# Autodesk Inventor assembly: smDriverStation-ver1-1111-2021
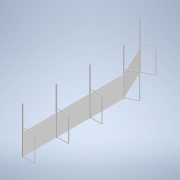
[picture p0: Inventor's stored thumbnail of the model, 180x180]
Saved by Autodesk Inventor 2021 (Build 250183000, 183)
## iProperties
Created: 2021-03-02
Part Number: smDriverStation-ver1-1111-2021
Document SubType Name: Assembly
Designer: CMurray
Author: CMurray
## Documents named in this file (3)
- F:\PHRC CADD 2021\2021 Game Design Challenge\Player Station\Assemblies\smDriverStation-ver1-1111-2021.iam
- F:\PHRC CADD 2021\2021 Game Design Challenge\Player Station\Parts\StationBase-ver2-1111-2021.ipt
- F:\PHRC CADD 2021\2021 Game Design Challenge\Player Station\Parts\StationDivider-ver1-1111-2021.iam
## Components (9 placed, 2 different names)
1. StationBase-ver2-1111-2021:2 — Mate:1, Flush:1, Flush:2, Mate:2, Flush:3, Flush:4, Flush:9, Flush:10
2. StationDivider-ver1-1111-2021:3 [sub-assembly] — Mate:1, Flush:1, Flush:2
3. StationDivider-ver1-1111-2021:4 [sub-assembly] — Mate:2, Flush:3, Flush:4, Mate:5
4. StationBase-ver2-1111-2021:3 — Flush:9, Flush:10, Mate:5, Flush:11, Flush:12
5. StationDivider-ver1-1111-2021:6 [sub-assembly] — Mate:6
6. StationBase-ver2-1111-2021:4 — Flush:11, Flush:12, Mate:6, Mate:7, Flush:13, Angle:1, Flush:14
7. StationDivider-ver1-1111-2021:7 [sub-assembly] — Mate:7, Flush:13, Mate:8, Angle:2
8. StationBase-ver2-1111-2021:5 — Mate:8, Angle:1, Flush:14, Mate:9, Flush:15, Flush:16
9. StationDivider-ver1-1111-2021:8 [sub-assembly] — Mate:9, Flush:15, Flush:16, Angle:2
## Relationships (24: Flush 14, Mate 8, Angle 2)
- Mate:1: StationBase-ver2-1111-2021:2 ↔ StationDivider-ver1-1111-2021:3
- Flush:1: StationBase-ver2-1111-2021:2 ↔ StationDivider-ver1-1111-2021:3
- Flush:2: StationBase-ver2-1111-2021:2 ↔ StationDivider-ver1-1111-2021:3
- Mate:2: StationBase-ver2-1111-2021:2 ↔ StationDivider-ver1-1111-2021:4
- Flush:3: StationBase-ver2-1111-2021:2 ↔ StationDivider-ver1-1111-2021:4
- Flush:4: StationBase-ver2-1111-2021:2 ↔ StationDivider-ver1-1111-2021:4
- [Mate]: StationBase-ver2-1111-2021:3 ↔ StationDivider-ver1-1111-2021:6
- [Flush]: StationBase-ver2-1111-2021:3 ↔ StationDivider-ver1-1111-2021:6
- [Flush]: StationBase-ver2-1111-2021:3 ↔ StationDivider-ver1-1111-2021:6
- Flush:9: StationBase-ver2-1111-2021:2 ↔ StationBase-ver2-1111-2021:3
- Flush:10: StationBase-ver2-1111-2021:2 ↔ StationBase-ver2-1111-2021:3
- Mate:5: StationDivider-ver1-1111-2021:4 ↔ StationBase-ver2-1111-2021:3
- Flush:11: StationBase-ver2-1111-2021:3 ↔ StationBase-ver2-1111-2021:4
- Flush:12: StationBase-ver2-1111-2021:3 ↔ StationBase-ver2-1111-2021:4
- Mate:6: StationDivider-ver1-1111-2021:6 ↔ StationBase-ver2-1111-2021:4
- Mate:7: StationBase-ver2-1111-2021:4 ↔ StationDivider-ver1-1111-2021:7
- Flush:13: StationBase-ver2-1111-2021:4 ↔ StationDivider-ver1-1111-2021:7
- Mate:8: StationDivider-ver1-1111-2021:7 ↔ StationBase-ver2-1111-2021:5
- Angle:1 (-25 deg): StationBase-ver2-1111-2021:4 ↔ StationBase-ver2-1111-2021:5
- Flush:14: StationBase-ver2-1111-2021:4 ↔ StationBase-ver2-1111-2021:5
- Mate:9: StationBase-ver2-1111-2021:5 ↔ StationDivider-ver1-1111-2021:8
- Flush:15: StationBase-ver2-1111-2021:5 ↔ StationDivider-ver1-1111-2021:8
- Flush:16: StationBase-ver2-1111-2021:5 ↔ StationDivider-ver1-1111-2021:8
- Angle:2 (0 deg): StationDivider-ver1-1111-2021:7 ↔ StationDivider-ver1-1111-2021:8
## Named parameters: d8_d4 = 0 mm, d9_d5 = 0 mm, d10_d6 = 0 mm
